# Autodesk Inventor assembly: UBG-StraightKick
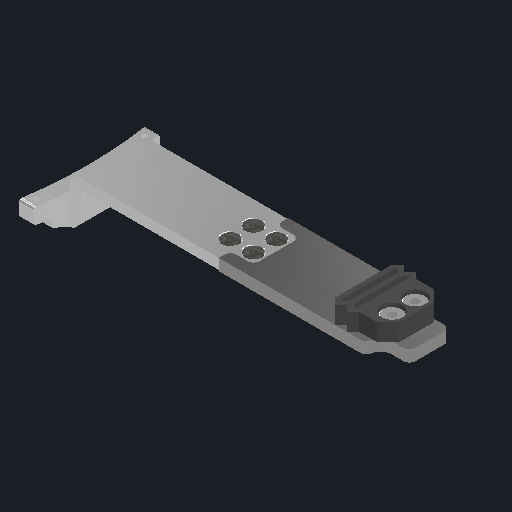
[picture p0: Inventor's stored thumbnail of the model, 512x512]
Saved by Autodesk Inventor 2025.2 (Build 292293000, 293)
## iProperties
Created: 2024-11-07
Part Number: UBG-StraightKick
Document SubType Name: Assembly
Designer: Fabian
Author: Fabian
## Documents named in this file (6)
- C:\Users\Faabs\Desktop\HBG v2025\Unterbaugruppen\UBG-Schussbauteile\UBG-Schuss\UBG-Schuss.iam
- C:\Users\Faabs\Desktop\HBG v2025\Unterbaugruppen\UBG-Schussbauteile\UBG-Schuss\Bauteile\Tauchkern.ipt
- C:\Users\Faabs\Desktop\HBG v2025\Unterbaugruppen\UBG-Schussbauteile\UBG-Schuss\Bauteile\SchussEisen.ipt
- C:\Users\Faabs\Desktop\HBG v2025\Verbindungselemente\ISO 10642\ISO 10642  - M3  x  4.ipt
- C:\Users\Faabs\Desktop\HBG v2025\Unterbaugruppen\UBG-Schussbauteile\UBG-Schuss\Bauteile\SchussDämpfung.ipt
- C:\Users\Faabs\Desktop\HBG v2025\Verbindungselemente\DIN 7984\DIN 7984 - M4 x 6.ipt
## Components (9 placed, 5 different names)
1. Tauchkern:1 — Passend:8, Passend:9, Passend:10, Fluchtend:1, Fluchtend:2, Fluchtend:3, Fluchtend:4
2. SchussEisen:1 — Passend:8, Passend:9, Passend:10, Passend:11, Passend:12, Passend:13, Passend:14, Passend:15, Passend:16, Passend:17
3. SchussDämpfung:1 — Passend:15, Passend:16, Passend:17, Einfügen:1, Einfügen:2
4. DIN EN ISO 10642 M3  x  8:5 — Passend:12, Fluchtend:1
5. DIN EN ISO 10642 M3  x  8:4 — Passend:13, Fluchtend:3
6. DIN EN ISO 10642 M3  x  8:3 — Passend:14, Fluchtend:4
7. DIN EN ISO 10642 M3  x  8:2 — Passend:11, Fluchtend:2
8. DIN 7984 M4 x 6:1 — Einfügen:2
9. DIN 7984 M4 x 6:2 — Einfügen:1
## Relationships (16: Mate 10, Flush 4, Insert 2)
- Passend:8 [Mate] (0.4 mm): Tauchkern:1 ↔ SchussEisen:1
- Passend:9 [Mate]: Tauchkern:1 ↔ SchussEisen:1
- Passend:10 [Mate]: Tauchkern:1 ↔ SchussEisen:1
- Passend:11 [Mate]: SchussEisen:1 ↔ DIN EN ISO 10642 M3  x  8:2
- Passend:12 [Mate]: SchussEisen:1 ↔ DIN EN ISO 10642 M3  x  8:5
- Passend:13 [Mate]: SchussEisen:1 ↔ DIN EN ISO 10642 M3  x  8:4
- Passend:14 [Mate]: SchussEisen:1 ↔ DIN EN ISO 10642 M3  x  8:3
- Fluchtend:1 [Flush]: Tauchkern:1 ↔ DIN EN ISO 10642 M3  x  8:5
- Fluchtend:2 [Flush]: Tauchkern:1 ↔ DIN EN ISO 10642 M3  x  8:2
- Fluchtend:3 [Flush]: Tauchkern:1 ↔ DIN EN ISO 10642 M3  x  8:4
- Fluchtend:4 [Flush]: Tauchkern:1 ↔ DIN EN ISO 10642 M3  x  8:3
- Passend:15 [Mate]: SchussEisen:1 ↔ SchussDämpfung:1
- Passend:16 [Mate]: SchussEisen:1 ↔ SchussDämpfung:1
- Passend:17 [Mate]: SchussEisen:1 ↔ SchussDämpfung:1
- Einfügen:1 [Insert]: SchussDämpfung:1 ↔ DIN 7984 M4 x 6:2
- Einfügen:2 [Insert]: SchussDämpfung:1 ↔ DIN 7984 M4 x 6:1
